# Autodesk Inventor assembly: Assembly2
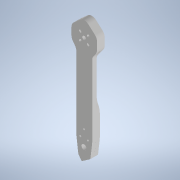
[picture p0: Inventor's stored thumbnail of the model, 180x180]
Saved by Autodesk Inventor 2020 (Build 240168000, 168)
## iProperties
Created: 2022-08-12
Part Number: Assembly2
Document SubType Name: Assembly
Designer: Steven
Author: Steven
## Documents named in this file (3)
- Y:\FPV drone stuff\0 Street League\Frames\experimental-quad-frames\Kauri assm\OG kauri mods\Assembly2.iam
- Y:\FPV drone stuff\0 Street League\Frames\experimental-quad-frames\Kauri assm\OG kauri mods\og kauri arm.ipt
- Y:\FPV drone stuff\0 Street League\Frames\experimental-quad-frames\Kauri assm\OG kauri mods\froggy kauri arm.ipt
## Components (2 placed, 2 different names)
1. og kauri arm:1 — Mate:1, Mate:2, Mate:3, Flush:1, Flush:2, Flush:3
2. froggy kauri arm:1 — Mate:1, Mate:2, Mate:3
## Relationships (6: Mate 3, Flush 3)
- Mate:1: og kauri arm:1 ↔ froggy kauri arm:1
- Mate:2: og kauri arm:1 ↔ froggy kauri arm:1
- Mate:3: og kauri arm:1 ↔ froggy kauri arm:1
- Flush:1: og kauri arm:1
- Flush:2: og kauri arm:1
- Flush:3: og kauri arm:1
